# Autodesk Inventor assembly: Helicopter_INSA_150
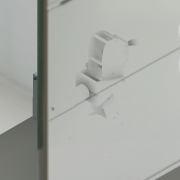
[picture p0: Inventor's stored thumbnail of the model, 180x180]
Saved by Autodesk Inventor 2016 SP1 (Build 200210100, 210)
## iProperties
Created: 2016-01-21
Part Number: Helicopter_INSA_150
Document SubType Name: Assembly
Designer: sd
Mass: 534.122 g
Surface Area: 1113.67 cm^2
Volume: 178.667 cm^3
Density: 2.98947 g/cm^3
Author: sd
## Documents named in this file (30)
- D:\Users\dimercur\Documents\SVN\projets-gei\Helicoptere_INSA_150\Helicopter_INSA_150.iam
- D:\Users\dimercur\Documents\SVN\projets-gei\Helicoptere_INSA_150\Cote_Gauche.ipt
- D:\Users\dimercur\Documents\SVN\projets-gei\Helicoptere_INSA_150\Cote_Droit.ipt
- D:\Users\dimercur\Documents\SVN\projets-gei\Helicoptere_INSA_150\Entretoise-50mm.ipt
- D:\Users\dimercur\Documents\SVN\projets-gei\Helicoptere_INSA_150\Nidec_DMN29.ipt
- D:\Users\dimercur\Documents\SVN\projets-gei\Helicoptere_INSA_150\Fixation_moteur.ipt
- D:\Users\dimercur\Documents\SVN\projets-gei\Helicoptere_INSA_150\Nidec_DMN37.ipt
- D:\Users\dimercur\Documents\SVN\projets-gei\Helicoptere_INSA_150\Helice 7x3.ipt
- D:\Users\dimercur\Documents\SVN\projets-gei\Helicoptere_INSA_150\Helice 4.5x4.5.ipt
- D:\Users\dimercur\Documents\SVN\projets-gei\Helicoptere_INSA_150\Potence.ipt
- D:\Users\dimercur\Documents\SVN\projets-gei\Helicoptere_INSA_150\Roulement.ipt
- D:\Users\dimercur\Documents\SVN\projets-gei\Helicoptere_INSA_150\Bague.ipt
- D:\Users\dimercur\Documents\SVN\projets-gei\Helicoptere_INSA_150\Vis-Pivot.ipt
- D:\Users\dimercur\Documents\SVN\projets-gei\Helicoptere_INSA_150\Vishay-157.ipt
- D:\Users\dimercur\Documents\SVN\projets-gei\Helicoptere_INSA_150\Fixation-potar.ipt
- D:\Users\dimercur\Documents\SVN\projets-gei\Helicoptere_INSA_150\Equerre-Potar.ipt
- D:\Users\dimercur\Documents\SVN\projets-gei\Helicoptere_INSA_150\SRC022.ipt
- D:\Users\dimercur\Documents\SVN\projets-gei\Helicoptere_INSA_150\Mat.ipt
- D:\Users\dimercur\Documents\SVN\projets-gei\Helicoptere_INSA_150\Base.ipt
- D:\Users\dimercur\Documents\SVN\projets-gei\Helicoptere_INSA_150\Bouchon PVC.ipt
- D:\Users\dimercur\Documents\SVN\projets-gei\Helicoptere_INSA_150\Raccord-Mat-Potence.ipt
- D:\Users\dimercur\Documents\Inventor\Content Center Files\R2016\fr-FR\ISO 4762(2)\ISO 4762 - M3 x 10ISO.ipt
- D:\Users\dimercur\Documents\Inventor\Content Center Files\R2016\fr-FR\ANSI B18.3.1M(1)\ANSI B18.3.1M - M3x0,5 x 55(2).ipt
- D:\Users\dimercur\Documents\Inventor\Content Center Files\R2016\fr-FR\ISO 4035(2)\ISO 4035 - M3,5 - ISO.ipt
- D:\Users\dimercur\Documents\Inventor\Content Center Files\R2016\fr-FR\DIN 7984\DIN 7984 - M3 x 5.ipt
- D:\Users\dimercur\Documents\Inventor\Content Center Files\R2016\fr-FR\DIN 7985 (Z)\DIN 7985 (Z) - M2x2-Z.ipt
- D:\Users\dimercur\Documents\Inventor\Content Center Files\R2016\fr-FR\ISO 4762(2)\ISO 4762 - M5 x 8ISO.ipt
- D:\Users\dimercur\Documents\Inventor\Content Center Files\R2016\fr-FR\ISO 4762(2)\ISO 4762 - M3 x 5ISO.ipt
- D:\Users\dimercur\Documents\Inventor\Content Center Files\R2016\fr-FR\ISO 7436(4)\ISO 7436 - M3,5 x 4 - DIN EN.ipt
- D:\Users\dimercur\Documents\SVN\projets-gei\Helicoptere_INSA_150\Pied.ipt
## Components (67 placed, 29 different names)
1. Cote_Gauche:1 — Logement:3, Logement:4, Logement:5, Logement:6, Logement:8, Logement:9, Placage:8, Placage:16, Placage:17, Placage:29, Placage:34, Logement:34, Logement:37, Logement:38, Logement:39, Logement:40, Logement:42, Logement:43, Logement:44, Logement:58, Logement:59, Logement:60
2. Cote_Droit:1 — Logement:12, Logement:13, Logement:33, Placage:1, Placage:14, Placage:15, Placage:30, Placage:41, Logement:45, Logement:47, Logement:48, Logement:49, Logement:51, Logement:52, Logement:53, Logement:54, Logement:55, Logement:57, Logement:64, Logement:65
3. Entretoise-50mm:3 — Logement:3
4. Entretoise-50mm:4 — Logement:4
5. Entretoise-50mm:5 — Logement:5, Logement:13
6. Entretoise-50mm:6 — Logement:6
7. Entretoise-50mm:8 — Logement:8, Logement:12
8. Entretoise-50mm:9 — Logement:9
9. Nidec_DMN29:1 — Logement:33, Placage:1, Placage:21, Affleurement:2
10. Fixation_moteur:1 — Placage:8, Placage:11, Placage:12, Placage:13, Logement:61, Logement:62, Logement:63, Placage:76, Placage:77
11. Nidec_DMN37:1 — Placage:11, Placage:12, Placage:13, Placage:20, Affleurement:1
12. Entretoise-50mm:10 — Placage:14, Placage:16
13. Entretoise-50mm:11 — Placage:15, Placage:17
14. Helice 7x3:1 — Placage:20, Affleurement:1
15. Helice 4.5x4.5:1 — Placage:21, Affleurement:2
16. Potence:1 — Placage:24, Placage:25, Placage:26, Placage:28, Placage:35, Placage:46, Placage:49, Placage:60
17. Roulement:1 — Placage:24, Placage:25, Placage:44
18. Roulement:2 — Placage:26, Placage:27, Placage:31, Placage:34, Placage:35, Placage:38, Placage:39
19. Bague:1 — Placage:28, Placage:30, Placage:40
20. Bague:2 — Placage:27, Placage:29, Placage:31
21. Vis-Pivot:1 — Placage:40, Placage:41, Placage:42, Placage:43, Placage:45
22. Vis-Pivot:2 — Placage:38, Placage:39
23. Vishay-157:1 — Placage:42, Placage:43, Placage:47
24. Fixation-potar:1 — Placage:44, Placage:45, Placage:65
25. Equerre-Potar:1 — Placage:46, Placage:47, Logement:69, Placage:66
26. SRC022:1 — Placage:49, Placage:58, Placage:59, Placage:60, Logement:66, Logement:67, Logement:68
27. Mat:1 — Placage:51, Placage:52, Placage:53, Placage:54, Placage:59
28. Base:1 — Placage:53, Placage:54, Placage:67, Placage:68, Placage:69, Placage:70, Placage:71, Placage:72, Placage:73, Placage:74, Placage:75
29. Bouchon PVC:1 — Placage:51, Placage:52, Placage:55, Placage:56, Placage:57
30. Raccord-Mat-Potence:1 — Placage:55, Placage:56, Placage:57, Placage:58, Placage:64
31. ISO 4762 M3 x 10:1 — Logement:34
32. ISO 4762 M3 x 10:4 — Logement:37
33. ISO 4762 M3 x 10:5 — Logement:38
34. ISO 4762 M3 x 10:6 — Logement:39
35. ISO 4762 M3 x 10:7 — Logement:40
36. ISO 4762 M3 x 10:9 — Logement:42
37. ISO 4762 M3 x 10:10 — Logement:43
38. ISO 4762 M3 x 10:11 — Logement:44
39. ISO 4762 M3 x 10:12 — Logement:45
40. ISO 4762 M3 x 10:14 — Logement:47
41. ISO 4762 M3 x 10:15 — Logement:48
42. ISO 4762 M3 x 10:16 — Logement:49
43. ISO 4762 M3 x 10:18 — Logement:51
44. ISO 4762 M3 x 10:19 — Logement:52
45. ISO 4762 M3 x 10:20 — Logement:53
46. ISO 4762 M3 x 10:21 — Logement:54
47. Vis à tête percée - Métrique M3x0,5 x 55:1 — Logement:55, Placage:76
48. Vis à tête percée - Métrique M3x0,5 x 55:3 — Logement:57, Placage:77
49. ISO 4035 M3,5:1 — Logement:58
50. ISO 4035 M3,5:2 — Logement:59
51. ISO 4035 M3,5:3 — Logement:60
52. DIN 7984 M3 x 5:1 — Logement:61
53. DIN 7984 M3 x 5:2 — Logement:62
54. DIN 7984 M3 x 5:3 — Logement:63
55. DIN 7985 (Z) M2x2-Z:1 — Logement:64
56. DIN 7985 (Z) M2x2-Z:2 — Logement:65
57. ISO 4762 M5 x 8:1 — Logement:66
58. ISO 4762 M5 x 8:2 — Logement:67
59. ISO 4762 M5 x 8:3 — Logement:68
60. ISO 4762 M3 x 5:1 — Logement:69
61. DIN EN 27436 M3,5 x 4:1 — Placage:65
62. DIN EN 27436 M3,5 x 4:2 — Placage:64
63. DIN EN 27436 M3,5 x 4:3 — Placage:66
64. Pied:1 — Placage:69, Placage:75
65. Pied:2 — Placage:68, Placage:73
66. Pied:3 — Placage:67, Placage:71, Placage:72
67. Pied:4 — Placage:70, Placage:74
## Relationships (97: Mate 56, Insert 39, Flush 2)
- Logement:3 [Insert]: Cote_Gauche:1 ↔ Entretoise-50mm:3
- Logement:4 [Insert]: Cote_Gauche:1 ↔ Entretoise-50mm:4
- Logement:5 [Insert]: Cote_Gauche:1 ↔ Entretoise-50mm:5
- Logement:6 [Insert]: Cote_Gauche:1 ↔ Entretoise-50mm:6
- Logement:8 [Insert]: Cote_Gauche:1 ↔ Entretoise-50mm:8
- Logement:9 [Insert]: Cote_Gauche:1 ↔ Entretoise-50mm:9
- Logement:12 [Insert]: Cote_Droit:1 ↔ Entretoise-50mm:8
- Logement:13 [Insert]: Cote_Droit:1 ↔ Entretoise-50mm:5
- Logement:33 [Insert]: Cote_Droit:1 ↔ Nidec_DMN29:1
- Placage:1 [Mate]: Cote_Droit:1 ↔ Nidec_DMN29:1
- Placage:8 [Mate]: Cote_Gauche:1 ↔ Fixation_moteur:1
- Placage:11 [Mate]: Fixation_moteur:1 ↔ Nidec_DMN37:1
- Placage:12 [Mate]: Fixation_moteur:1 ↔ Nidec_DMN37:1
- Placage:13 [Mate]: Fixation_moteur:1 ↔ Nidec_DMN37:1
- Placage:14 [Mate]: Cote_Droit:1 ↔ Entretoise-50mm:10
- Placage:15 [Mate]: Cote_Droit:1 ↔ Entretoise-50mm:11
- Placage:16 [Mate]: Cote_Gauche:1 ↔ Entretoise-50mm:10
- Placage:17 [Mate]: Cote_Gauche:1 ↔ Entretoise-50mm:11
- Placage:20 [Mate]: Nidec_DMN37:1 ↔ Helice 7x3:1
- Affleurement:1 [Flush]: Nidec_DMN37:1 ↔ Helice 7x3:1
- Placage:21 [Mate]: Nidec_DMN29:1 ↔ Helice 4.5x4.5:1
- Affleurement:2 [Flush]: Nidec_DMN29:1 ↔ Helice 4.5x4.5:1
- Placage:24 [Mate]: Potence:1 ↔ Roulement:1
- Placage:25 [Mate]: Potence:1 ↔ Roulement:1
- Placage:26 [Mate]: Potence:1 ↔ Roulement:2
- Placage:27 [Mate]: Roulement:2 ↔ Bague:2
- Placage:28 [Mate]: Potence:1 ↔ Bague:1
- Placage:29 [Mate]: Cote_Gauche:1 ↔ Bague:2
- Placage:30 [Mate]: Cote_Droit:1 ↔ Bague:1
- Placage:31 [Mate]: Roulement:2 ↔ Bague:2
- Placage:34 [Mate]: Cote_Gauche:1 ↔ Roulement:2
- Placage:35 [Mate]: Potence:1 ↔ Roulement:2
- Placage:38 [Mate]: Roulement:2 ↔ Vis-Pivot:2
- Placage:39 [Mate]: Roulement:2 ↔ Vis-Pivot:2
- Placage:40 [Mate]: Bague:1 ↔ Vis-Pivot:1
- Placage:41 [Mate]: Cote_Droit:1 ↔ Vis-Pivot:1
- Placage:42 [Mate]: Vis-Pivot:1 ↔ Vishay-157:1
- Placage:43 [Mate]: Vis-Pivot:1 ↔ Vishay-157:1
- Placage:44 [Mate]: Roulement:1 ↔ Fixation-potar:1
- Placage:45 [Mate]: Vis-Pivot:1 ↔ Fixation-potar:1
- Placage:46 [Mate]: Potence:1 ↔ Equerre-Potar:1
- Placage:47 [Mate]: Vishay-157:1 ↔ Equerre-Potar:1
- Placage:49 [Mate]: Potence:1 ↔ SRC022:1
- Placage:51 [Mate]: Mat:1 ↔ Bouchon PVC:1
- Placage:52 [Mate]: Mat:1 ↔ Bouchon PVC:1
- Placage:53 [Mate]: Mat:1 ↔ Base:1
- Placage:54 [Mate]: Mat:1 ↔ Base:1
- Placage:55 [Mate]: Bouchon PVC:1 ↔ Raccord-Mat-Potence:1
- Placage:56 [Mate]: Bouchon PVC:1 ↔ Raccord-Mat-Potence:1
- Placage:57 [Mate]: Bouchon PVC:1 ↔ Raccord-Mat-Potence:1
- Placage:58 [Mate] (1 mm): SRC022:1 ↔ Raccord-Mat-Potence:1
- Placage:59 [Mate]: SRC022:1 ↔ Mat:1
- Placage:60 [Mate]: Potence:1 ↔ SRC022:1
- Logement:34 [Insert]: Cote_Gauche:1 ↔ ISO 4762 M3 x 10:1
- Logement:37 [Insert]: Cote_Gauche:1 ↔ ISO 4762 M3 x 10:4
- Logement:38 [Insert]: Cote_Gauche:1 ↔ ISO 4762 M3 x 10:5
- Logement:39 [Insert]: Cote_Gauche:1 ↔ ISO 4762 M3 x 10:6
- Logement:40 [Insert]: Cote_Gauche:1 ↔ ISO 4762 M3 x 10:7
- Logement:42 [Insert]: Cote_Gauche:1 ↔ ISO 4762 M3 x 10:9
- Logement:43 [Insert]: Cote_Gauche:1 ↔ ISO 4762 M3 x 10:10
- Logement:44 [Insert]: Cote_Gauche:1 ↔ ISO 4762 M3 x 10:11
- Logement:45 [Insert]: Cote_Droit:1 ↔ ISO 4762 M3 x 10:12
- Logement:47 [Insert]: Cote_Droit:1 ↔ ISO 4762 M3 x 10:14
- Logement:48 [Insert]: Cote_Droit:1 ↔ ISO 4762 M3 x 10:15
- Logement:49 [Insert]: Cote_Droit:1 ↔ ISO 4762 M3 x 10:16
- Logement:51 [Insert]: Cote_Droit:1 ↔ ISO 4762 M3 x 10:18
- Logement:52 [Insert]: Cote_Droit:1 ↔ ISO 4762 M3 x 10:19
- Logement:53 [Insert]: Cote_Droit:1 ↔ ISO 4762 M3 x 10:20
- Logement:54 [Insert]: Cote_Droit:1 ↔ ISO 4762 M3 x 10:21
- Logement:55 [Insert]: Cote_Droit:1 ↔ Vis à tête percée - Métrique M3x0,5 x 55:1
- Logement:57 [Insert]: Cote_Droit:1 ↔ Vis à tête percée - Métrique M3x0,5 x 55:3
- Logement:58 [Insert]: Cote_Gauche:1 ↔ ISO 4035 M3,5:1
- Logement:59 [Insert]: Cote_Gauche:1 ↔ ISO 4035 M3,5:2
- Logement:60 [Insert]: Cote_Gauche:1 ↔ ISO 4035 M3,5:3
- Logement:61 [Insert]: Fixation_moteur:1 ↔ DIN 7984 M3 x 5:1
- Logement:62 [Insert]: Fixation_moteur:1 ↔ DIN 7984 M3 x 5:2
- Logement:63 [Insert]: Fixation_moteur:1 ↔ DIN 7984 M3 x 5:3
- Logement:64 [Insert]: Cote_Droit:1 ↔ DIN 7985 (Z) M2x2-Z:1
- Logement:65 [Insert]: Cote_Droit:1 ↔ DIN 7985 (Z) M2x2-Z:2
- Logement:66 [Insert]: SRC022:1 ↔ ISO 4762 M5 x 8:1
- Logement:67 [Insert]: SRC022:1 ↔ ISO 4762 M5 x 8:2
- Logement:68 [Insert]: SRC022:1 ↔ ISO 4762 M5 x 8:3
- Logement:69 [Insert]: Equerre-Potar:1 ↔ ISO 4762 M3 x 5:1
- Placage:64 [Mate]: Raccord-Mat-Potence:1 ↔ DIN EN 27436 M3,5 x 4:2
- Placage:65 [Mate]: Fixation-potar:1 ↔ DIN EN 27436 M3,5 x 4:1
- Placage:66 [Mate]: Equerre-Potar:1 ↔ DIN EN 27436 M3,5 x 4:3
- Placage:67 [Mate]: Base:1 ↔ Pied:3
- Placage:68 [Mate]: Base:1 ↔ Pied:2
- Placage:69 [Mate]: Base:1 ↔ Pied:1
- Placage:70 [Mate]: Base:1 ↔ Pied:4
- Placage:71 [Mate]: Base:1 ↔ Pied:3
- Placage:72 [Mate]: Base:1 ↔ Pied:3
- Placage:73 [Mate]: Base:1 ↔ Pied:2
- Placage:74 [Mate]: Base:1 ↔ Pied:4
- Placage:75 [Mate]: Base:1 ↔ Pied:1
- Placage:76 [Mate]: Fixation_moteur:1 ↔ Vis à tête percée - Métrique M3x0,5 x 55:1
- Placage:77 [Mate]: Fixation_moteur:1 ↔ Vis à tête percée - Métrique M3x0,5 x 55:3
